# Autodesk Inventor assembly: Gantry 4x4
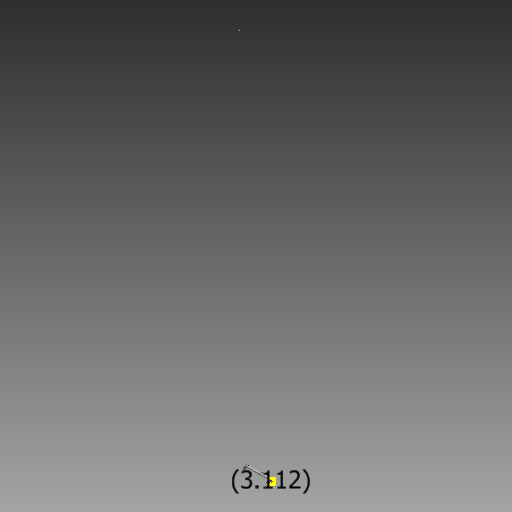
[picture p0: Inventor's stored thumbnail of the model, 512x512]
Saved by Autodesk Inventor 2019 (Build 230136000, 136)
## iProperties
Created: 2017-12-18
Part Number: Gantry 4x4
Document SubType Name: Assembly
Designer: torba
Author: torba
## Documents named in this file (21)
- C:\Users\torba\Nextcloud\Projects\Inventor\Plasma 5x10\Gantry 4x4.iam
- C:\Users\torba\OneDrive\Documents\Inventor\Plasma 5x10\3 x 3 TUBE .125 steel.ipt
- C:\Users\torba\OneDrive\Documents\Inventor\Plasma 5x10\4x.25 cold rolled steel.ipt
- C:\Users\torba\Nextcloud\Projects\Inventor\Plasma 5x10\gantry inner.ipt
- C:\Users\torba\OneDrive\Documents\Inventor\Plasma 5x10\1 x 3 tube .125.ipt
- C:\Users\torba\Nextcloud\Projects\Inventor\Plasma 5x10\Gantry Outer.ipt
- C:\Users\torba\Nextcloud\Projects\Inventor\Plasma 5x10\CPM-341x\CPM-_ _ _ _ - 3411_-LS.ipt
- C:\Users\torba\Nextcloud\Projects\Inventor\Plasma 5x10\Gantry Side load assy.iam
- C:\Users\torba\Nextcloud\Projects\Inventor\Plasma 5x10\Servo Flange.ipt
- C:\Users\torba\Nextcloud\Projects\Inventor\Plasma 5x10\PSC1024 Gear (Simplified).ipt
- C:\Users\torba\Nextcloud\Projects\Inventor\Plasma 5x10\Bearing Assembly.iam
- C:\Users\torba\OneDrive\Documents\Inventor\Plasma 5x10\RSHC10XX00 Rack (Simplified).ipt
- C:\Users\torba\Nextcloud\Projects\Inventor\Plasma 5x10\Drag Chain End.ipt
- C:\Users\torba\Nextcloud\Projects\Inventor\Plasma 5x10\Gantry Chain Support.ipt
- C:\Users\torba\Nextcloud\Projects\Inventor\Plasma 5x10\Limit Switch.ipt
- C:\Users\torba\Nextcloud\Projects\Inventor\Plasma 5x10\Limit Mount.ipt
- C:\Users\torba\Nextcloud\Projects\Inventor\Plasma 5x10\3 x 3 TUBE .125 steel\3 x 3 TUBE .125 steel-69.75.ipt
- C:\Users\torba\Nextcloud\Projects\Inventor\Plasma 5x10\1 x 3 tube .125\1 x 3 tube .125-62.ipt
- C:\Users\torba\Nextcloud\Projects\Inventor\Plasma 5x10\4x.25 cold rolled steel\4x.25 cold rolled steel-61.ipt
- C:\Users\torba\Nextcloud\Projects\Inventor\Plasma 5x10\RSHC10XX00 Rack (Simplified)\RSHC10XX00 Rack (Simplified)-56.5.ipt
- C:\Users\torba\Nextcloud\Projects\Inventor\Plasma 5x10\Y reduction Assy.iam
## Components (39 placed, 16 different names)
1. 3 x 3 TUBE .125 steel-69.75:2 — Mate:2, Mate:3, Mate:6, Mate:7, Flush:4, Flush:5, Mate:76, Mate:77, Mate:81, Mate:132, Mate:138, Flush:20, Mate:166, Flush:40, Angle:2
2. 4x.25 cold rolled steel-61:1 — Mate:166, Flush:40, Mate:169
3. gantry inner:1 — Mate:3, Mate:6, Mate:111, Mate:112, Mate:113, Mate:125, Mate:127, Mate:128, Flush:25, Mate:157, Mate:167, Mate:169
4. gantry inner:2 — Mate:2, Mate:7, Mate:22, Mate:23, Flush:3, Mate:117, Mate:118, Mate:119, Mate:121, Mate:122, Mate:123, Mate:139, Mate:150, Flush:26, Mate:156, Mate:168
5. 1 x 3 tube .125-62:1 — Mate:22, Mate:23, Flush:3, Mate:149, Flush:22
6. Gantry Outer:1 — Flush:5, Mate:76, Mate:77, Mate:115, Mate:116, Mate:120, Mate:124, Mate:133, Mate:135, Mate:137, Mate:140, Mate:141, Mate:153, Flush:23, Flush:24, Mate:168, Mate:173, Mate:174
7. Gantry Outer:2 — Flush:4, Mate:81, Mate:110, Mate:114, Mate:126, Mate:129, Mate:131, Mate:132, Mate:134, Mate:148, Angle:1, Mate:167
8. Bearing Assembly:1 [sub-assembly] — Mate:110, Mate:129
9. Bearing Assembly:2 [sub-assembly] — Mate:113, Mate:125
10. Bearing Assembly:3 [sub-assembly] — Mate:111, Mate:128
11. Bearing Assembly:4 [sub-assembly] — Mate:116, Mate:120
12. Bearing Assembly:5 [sub-assembly] — Mate:112, Mate:127
13. Bearing Assembly:6 [sub-assembly] — Mate:117, Mate:122
14. Bearing Assembly:7 [sub-assembly] — Mate:118, Mate:123
15. Bearing Assembly:8 [sub-assembly] — Mate:119, Mate:121
16. Bearing Assembly:9 [sub-assembly] — Mate:114, Mate:126
17. Bearing Assembly:10 [sub-assembly] — Mate:115, Mate:124
18. RSHC10XX00 Rack (Simplified)-56.5:1 — Mate:138, Flush:20, Mate:139
19. Gantry Side load assy:5 [sub-assembly] — Flush:15, Flush:19, Mate:133, Mate:141, Mate:160, Flush:30, Flush:34
20. Gantry Side load assy:6 [sub-assembly] — Flush:16, Flush:17, Flush:18, Mate:134, Flush:33
21. Gantry Side load assy:7 [sub-assembly] — Flush:17, Flush:18, Mate:135, Mate:137, Mate:140, Flush:31
22. Gantry Side load assy:8 [sub-assembly] — Flush:15, Flush:16, Flush:19, Mate:131, Mate:161, Flush:32, Flush:35
23. CPM-_ _ _ _ - 3411_-LS:2 — Angle:1
24. Servo Flange:2 — Mate:148
25. PSC1024 Gear (Simplified):2
26. Drag Chain End:1 — Mate:149, Flush:22, Mate:150
27. Drag Chain End:2 — Mate:170, Mate:171, Mate:172
28. Gantry Chain Support:1 — Mate:153, Flush:23, Flush:24, Mate:170, Mate:171, Mate:172
29. Limit Switch:1 — Flush:25, Mate:157
30. Limit Switch:2 — Flush:26, Mate:156
31. Limit Mount:1 — Flush:27, Mate:159, Mate:161, Flush:32, Flush:35, Mate:164, Flush:37
32. Limit Mount:2 — Flush:27, Flush:28, Mate:159, Flush:33, Mate:165, Flush:36
33. Limit Mount:3 — Flush:28, Flush:29, Mate:158, Mate:160, Flush:30, Flush:34, Mate:162, Flush:39
34. Limit Mount:4 — Flush:29, Mate:158, Flush:31, Mate:163, Flush:38
35. Limit Switch:3 — Mate:165, Flush:36
36. Limit Switch:4 — Mate:164, Flush:37
37. Limit Switch:5 — Mate:163, Flush:38
38. Limit Switch:6 — Mate:162, Flush:39
39. Y reduction Assy:1 [sub-assembly] — Mate:173, Mate:174, Angle:2
## Relationships (97: Mate 66, Flush 29, Angle 2)
- Mate:2: 3 x 3 TUBE .125 steel-69.75:2 ↔ gantry inner:2
- Mate:3: 3 x 3 TUBE .125 steel-69.75:2 ↔ gantry inner:1
- Mate:6: 3 x 3 TUBE .125 steel-69.75:2 ↔ gantry inner:1
- Mate:7: 3 x 3 TUBE .125 steel-69.75:2 ↔ gantry inner:2
- Mate:22: gantry inner:2 ↔ 1 x 3 tube .125-62:1
- Mate:23: gantry inner:2 ↔ 1 x 3 tube .125-62:1
- Flush:3 (-6.35 mm): gantry inner:2 ↔ 1 x 3 tube .125-62:1
- Flush:4 (9.525 mm): 3 x 3 TUBE .125 steel-69.75:2 ↔ Gantry Outer:2
- Flush:5 (9.525 mm): 3 x 3 TUBE .125 steel-69.75:2 ↔ Gantry Outer:1
- Mate:76: 3 x 3 TUBE .125 steel-69.75:2 ↔ Gantry Outer:1
- Mate:77: 3 x 3 TUBE .125 steel-69.75:2 ↔ Gantry Outer:1
- Mate:81: 3 x 3 TUBE .125 steel-69.75:2 ↔ Gantry Outer:2
- Mate:110: Gantry Outer:2 ↔ Bearing Assembly:1
- Mate:111: gantry inner:1 ↔ Bearing Assembly:3
- Mate:112: gantry inner:1 ↔ Bearing Assembly:5
- Mate:113: gantry inner:1 ↔ Bearing Assembly:2
- Mate:114: Gantry Outer:2 ↔ Bearing Assembly:9
- Mate:115: Gantry Outer:1 ↔ Bearing Assembly:10
- Mate:116: Gantry Outer:1 ↔ Bearing Assembly:4
- Mate:117: gantry inner:2 ↔ Bearing Assembly:6
- Mate:118: gantry inner:2 ↔ Bearing Assembly:7
- Mate:119: gantry inner:2 ↔ Bearing Assembly:8
- Mate:120: Gantry Outer:1 ↔ Bearing Assembly:4
- Mate:121: gantry inner:2 ↔ Bearing Assembly:8
- Mate:122: gantry inner:2 ↔ Bearing Assembly:6
- Mate:123: gantry inner:2 ↔ Bearing Assembly:7
- Mate:124: Gantry Outer:1 ↔ Bearing Assembly:10
- Mate:125: gantry inner:1 ↔ Bearing Assembly:2
- Mate:126: Gantry Outer:2 ↔ Bearing Assembly:9
- Mate:127: gantry inner:1 ↔ Bearing Assembly:5
- Mate:128: gantry inner:1 ↔ Bearing Assembly:3
- Mate:129: Gantry Outer:2 ↔ Bearing Assembly:1
- Flush:15: Gantry Side load assy:5 ↔ Gantry Side load assy:8
- Flush:16: Gantry Side load assy:6 ↔ Gantry Side load assy:8
- Flush:17: Gantry Side load assy:6 ↔ Gantry Side load assy:7
- Flush:18: Gantry Side load assy:6 ↔ Gantry Side load assy:7
- Flush:19: Gantry Side load assy:5 ↔ Gantry Side load assy:8
- Mate:131: Gantry Outer:2 ↔ Gantry Side load assy:8
- Mate:132: 3 x 3 TUBE .125 steel-69.75:2 ↔ Gantry Outer:2
- Mate:133: Gantry Outer:1 ↔ Gantry Side load assy:5
- Mate:134: Gantry Outer:2 ↔ Gantry Side load assy:6
- Mate:135: Gantry Outer:1 ↔ Gantry Side load assy:7
- Mate:137 (-19.0246 mm): Gantry Outer:1 ↔ Gantry Side load assy:7
- Mate:138: 3 x 3 TUBE .125 steel-69.75:2 ↔ RSHC10XX00 Rack (Simplified)-56.5:1
- Flush:20 (3.175 mm): 3 x 3 TUBE .125 steel-69.75:2 ↔ RSHC10XX00 Rack (Simplified)-56.5:1
- Mate:139 (57.15 mm): gantry inner:2 ↔ RSHC10XX00 Rack (Simplified)-56.5:1
- Mate:140: Gantry Outer:1 ↔ Gantry Side load assy:7
- Mate:141: Gantry Outer:1 ↔ Gantry Side load assy:5
- [Mate]: CPM-_ _ _ _ - 3411_-LS:2 ↔ Servo Flange:2
- [Mate]: CPM-_ _ _ _ - 3411_-LS:2 ↔ Servo Flange:2
- [Mate]: CPM-_ _ _ _ - 3411_-LS:2 ↔ Servo Flange:2
- [Flush]: CPM-_ _ _ _ - 3411_-LS:2 ↔ PSC1024 Gear (Simplified):2
- [Mate]: CPM-_ _ _ _ - 3411_-LS:2 ↔ PSC1024 Gear (Simplified):2
- Mate:148: Gantry Outer:2 ↔ Servo Flange:2
- Angle:1 (225 deg): Gantry Outer:2 ↔ CPM-_ _ _ _ - 3411_-LS:2
- Mate:149: 1 x 3 tube .125-62:1 ↔ Drag Chain End:1
- Flush:22 (-11.8999 mm): 1 x 3 tube .125-62:1 ↔ Drag Chain End:1
- Mate:150 (609.6 mm): gantry inner:2 ↔ Drag Chain End:1
- Mate:153: Gantry Outer:1 ↔ Gantry Chain Support:1
- Flush:23 (-25.4 mm): Gantry Outer:1 ↔ Gantry Chain Support:1
- Flush:24 (-6.35 mm): Gantry Outer:1 ↔ Gantry Chain Support:1
- Flush:25 (25.4 mm): gantry inner:1 ↔ Limit Switch:1
- Flush:26 (-25.4 mm): gantry inner:2 ↔ Limit Switch:2
- Mate:156: gantry inner:2 ↔ Limit Switch:2
- Mate:157: gantry inner:1 ↔ Limit Switch:1
- Flush:27: Limit Mount:1 ↔ Limit Mount:2
- Flush:28: Limit Mount:2 ↔ Limit Mount:3
- Flush:29: Limit Mount:3 ↔ Limit Mount:4
- Mate:158: Limit Mount:3 ↔ Limit Mount:4
- Mate:159: Limit Mount:1 ↔ Limit Mount:2
- Mate:160: Gantry Side load assy:5 ↔ Limit Mount:3
- Mate:161: Gantry Side load assy:8 ↔ Limit Mount:1
- Flush:30 (31.75 mm): Gantry Side load assy:5 ↔ Limit Mount:3
- Flush:31 (31.75 mm): Gantry Side load assy:7 ↔ Limit Mount:4
- Flush:32 (31.75 mm): Gantry Side load assy:8 ↔ Limit Mount:1
- Flush:33 (31.75 mm): Gantry Side load assy:6 ↔ Limit Mount:2
- Flush:34 (-45.466 mm): Gantry Side load assy:5 ↔ Limit Mount:3
- Flush:35 (45.466 mm): Gantry Side load assy:8 ↔ Limit Mount:1
- Mate:162: Limit Mount:3 ↔ Limit Switch:6
- Mate:163: Limit Mount:4 ↔ Limit Switch:5
- Mate:164: Limit Mount:1 ↔ Limit Switch:4
- Mate:165: Limit Mount:2 ↔ Limit Switch:3
- Flush:36 (-25.4 mm): Limit Mount:2 ↔ Limit Switch:3
- Flush:37 (-25.4 mm): Limit Mount:1 ↔ Limit Switch:4
- Flush:38 (-25.4 mm): Limit Mount:4 ↔ Limit Switch:5
- Flush:39 (-25.4 mm): Limit Mount:3 ↔ Limit Switch:6
- Mate:166: 3 x 3 TUBE .125 steel-69.75:2 ↔ 4x.25 cold rolled steel-61:1
- Flush:40 (12.7 mm): 3 x 3 TUBE .125 steel-69.75:2 ↔ 4x.25 cold rolled steel-61:1
- Mate:167 (88.9 mm): gantry inner:1 ↔ Gantry Outer:2
- Mate:168 (88.9 mm): gantry inner:2 ↔ Gantry Outer:1
- Mate:169: 4x.25 cold rolled steel-61:1 ↔ gantry inner:1
- Mate:170: Drag Chain End:2 ↔ Gantry Chain Support:1
- Mate:171: Drag Chain End:2 ↔ Gantry Chain Support:1
- Mate:172: Drag Chain End:2 ↔ Gantry Chain Support:1
- Mate:173: Gantry Outer:1 ↔ Y reduction Assy:1
- Mate:174: Gantry Outer:1 ↔ Y reduction Assy:1
- Angle:2 (0 deg): 3 x 3 TUBE .125 steel-69.75:2 ↔ Y reduction Assy:1
## Named parameters: d182_d141 = 0 mm, d183_d142 = 0 mm, d184_d115 = 0 mm, d185_d117 = 0 mm, d186_d113 = 0 mm
